# Autodesk Inventor assembly: drillmotor
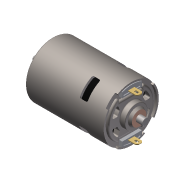
[picture p0: Inventor's stored thumbnail of the model, 180x180]
Saved by Autodesk Inventor 2015 (Build 190159000, 159)
## iProperties
Created: 2014-08-03
Part Number: drillmotor
Document SubType Name: Assembly
Designer: david
Author: david
## Documents named in this file (2)
- C:\SharedDrive\Dropbox\FAST Robotics\Products\FAST_ROVER\810002_ASY-FAST ROVER v2\813004_FAST ROVER v2 CHASSIS\813005_Hummer H2 Chassis\drill-motor-1.snapshot.1\drillmotor.iam
- C:\SharedDrive\Dropbox\FAST Robotics\Products\FAST_ROVER\810002_ASY-FAST ROVER v2\813004_FAST ROVER v2 CHASSIS\813005_Hummer H2 Chassis\drill-motor-1.snapshot.1\Imported Components\Motor\Motor.ipt
## Components (1 placed, 1 different names)
1. Motor:1 — Flush:1, Mate:1, Flush:2
## Relationships (3: Flush 2, Mate 1)
- Flush:1: Motor:1
- Mate:1: Motor:1
- Flush:2: Motor:1
